# Autodesk Inventor assembly: Gym Setup
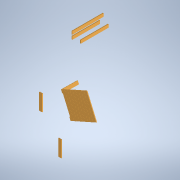
[picture p0: Inventor's stored thumbnail of the model, 180x180]
Saved by Autodesk Inventor 2021 (Build 250183000, 183)
## iProperties
Created: 2020-12-20
Part Number: Gym Setup
Document SubType Name: Assembly
Designer: Jawad
Author: Jawad
## Documents named in this file (4)
- E:\OneDrive - UNSW\Inventor-Designs\Gym Design\Gym Setup.iam
- E:\OneDrive - UNSW\Inventor-Designs\Gym Design\wooden beams.ipt
- E:\OneDrive - UNSW\Inventor-Designs\Gym Design\pull Up beams.ipt
- E:\OneDrive - UNSW\Inventor-Designs\Gym Design\Dip Beams.ipt
## Components (17 placed, 3 different names)
1. wooden beams:1 — Flush:10, Mate:9, Mate:10, Flush:14, Flush:15, Mate:16, Flush:19, Flush:21, Flush:23, Mate:17, Flush:24, Mate:18, Flush:25, Flush:26, Flush:27, Flush:28, Flush:29, Mate:19, Flush:30, Flush:31, Mate:20, Flush:32, Flush:33, Mate:21, Flush:34, Mate:22, Flush:35
2. wooden beams:2 — Mate:9, Flush:13, Flush:15, Mate:13, Flush:16, Flush:17, Mate:14, Flush:18, Mate:15, Flush:20, Flush:22
3. wooden beams:3 — Flush:9, Flush:10, Flush:12, Flush:13, Mate:12, Mate:13, Flush:16, Flush:17, Mate:14, Flush:18
4. wooden beams:4 — Mate:10, Flush:14, Mate:15, Mate:16, Flush:19, Flush:20, Flush:21, Flush:22, Flush:23, Mate:17
5. wooden beams:5 — Flush:6, Mate:8, Flush:7, Flush:8, Flush:11, Mate:11
6. wooden beams:6 — Flush:4, Flush:5, Mate:2, Flush:6, Mate:8, Flush:7
7. wooden beams:7 — Flush:8, Flush:9, Flush:11, Flush:12, Mate:11, Mate:12
8. wooden beams:8 — Flush:1, Mate:1, Flush:2, Flush:3
9. wooden beams:9 — Flush:1, Mate:1, Flush:2, Flush:3, Flush:4, Flush:5, Mate:2
10. pull Up beams:1
11. pull Up beams:2
12. pull Up beams:3
13. pull Up beams:4
14. Dip Beams:1 — Mate:20, Flush:32, Flush:33, Mate:21, Flush:34, Mate:22, Flush:35
15. Dip Beams:2
16. Dip Beams:3
17. Dip Beams:4 — Flush:24, Mate:18, Flush:25, Flush:26, Flush:27, Flush:28, Flush:29, Mate:19, Flush:30, Flush:31
## Relationships (52: Flush 35, Mate 17)
- Flush:1: wooden beams:8 ↔ wooden beams:9
- Mate:1: wooden beams:8 ↔ wooden beams:9
- Flush:2: wooden beams:8 ↔ wooden beams:9
- Flush:3: wooden beams:8 ↔ wooden beams:9
- Flush:4: wooden beams:6 ↔ wooden beams:9
- Flush:5: wooden beams:6 ↔ wooden beams:9
- Mate:2: wooden beams:6 ↔ wooden beams:9
- Flush:6: wooden beams:5 ↔ wooden beams:6
- Mate:8: wooden beams:5 ↔ wooden beams:6
- Flush:7: wooden beams:5 ↔ wooden beams:6
- Flush:8: wooden beams:5 ↔ wooden beams:7
- Flush:9: wooden beams:3 ↔ wooden beams:7
- Flush:10: wooden beams:1 ↔ wooden beams:3
- Mate:9: wooden beams:1 ↔ wooden beams:2
- Mate:10: wooden beams:1 ↔ wooden beams:4
- Flush:11: wooden beams:5 ↔ wooden beams:7
- Flush:12: wooden beams:3 ↔ wooden beams:7
- Flush:13: wooden beams:2 ↔ wooden beams:3
- Flush:14: wooden beams:1 ↔ wooden beams:4
- Flush:15: wooden beams:1 ↔ wooden beams:2
- Mate:11: wooden beams:5 ↔ wooden beams:7
- Mate:12: wooden beams:3 ↔ wooden beams:7
- Mate:13: wooden beams:2 ↔ wooden beams:3
- Flush:16: wooden beams:2 ↔ wooden beams:3
- Flush:17: wooden beams:2 ↔ wooden beams:3
- Mate:14: wooden beams:2 ↔ wooden beams:3
- Flush:18: wooden beams:2 ↔ wooden beams:3
- Mate:15: wooden beams:2 ↔ wooden beams:4
- Mate:16: wooden beams:1 ↔ wooden beams:4
- Flush:19: wooden beams:1 ↔ wooden beams:4
- Flush:20: wooden beams:2 ↔ wooden beams:4
- Flush:21: wooden beams:1 ↔ wooden beams:4
- Flush:22: wooden beams:2 ↔ wooden beams:4
- Flush:23: wooden beams:1 ↔ wooden beams:4
- Mate:17: wooden beams:1 ↔ wooden beams:4
- Flush:24: wooden beams:1 ↔ Dip Beams:4
- Mate:18: wooden beams:1 ↔ Dip Beams:4
- Flush:25: wooden beams:1 ↔ Dip Beams:4
- Flush:26: wooden beams:1 ↔ Dip Beams:4
- Flush:27: wooden beams:1 ↔ Dip Beams:4
- Flush:28: wooden beams:1 ↔ Dip Beams:4
- Flush:29: wooden beams:1 ↔ Dip Beams:4
- Mate:19: wooden beams:1 ↔ Dip Beams:4
- Flush:30: wooden beams:1 ↔ Dip Beams:4
- Flush:31: wooden beams:1 ↔ Dip Beams:4
- Mate:20: wooden beams:1 ↔ Dip Beams:1
- Flush:32: wooden beams:1 ↔ Dip Beams:1
- Flush:33: wooden beams:1 ↔ Dip Beams:1
- Mate:21: wooden beams:1 ↔ Dip Beams:1
- Flush:34: wooden beams:1 ↔ Dip Beams:1
- Mate:22: wooden beams:1 ↔ Dip Beams:1
- Flush:35: wooden beams:1 ↔ Dip Beams:1
